# Autodesk Inventor assembly: Mark2
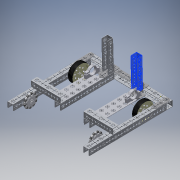
[picture p0: Inventor's stored thumbnail of the model, 180x180]
Saved by Autodesk Inventor 2017 (Build 210142000, 142)
## iProperties
Created: 2016-09-25
Part Number: Mark2
Document SubType Name: Assembly
Designer: Spartacles
Author: Spartacles
## Documents named in this file (14)
- C:\Users\Spartacles\Desktop\2016-Robot\2016launcher\Mark2.iam
- C:\Users\Spartacles\Desktop\2016-Robot\2016launcher\UTubes\Star3Tube.ipt
- C:\Users\Spartacles\Desktop\2016-Robot\2016launcher\UTubes\Star5Tube.ipt
- C:\Users\Spartacles\Desktop\2016-Robot\2016launcher\UTubes\Star7Tube.ipt
- C:\Users\Spartacles\Desktop\2016-Robot\Axle Hub\Axle hub thin.ipt
- C:\Users\Spartacles\Desktop\2016-Robot\Axel\Axel.ipt
- C:\Users\Spartacles\Desktop\2016-Robot\BlackWheels\4 Inch Wheel.ipt
- C:\Users\Spartacles\Desktop\2016-Robot\omni\3inch OmniWheel.iam
- C:\Users\Spartacles\Documents\Pitsco Education-739273\Pitsco Education-739273.ipt
- C:\Users\Spartacles\Documents\Pitsco Education-739272 (1)\Pitsco Education-739272.ipt
- C:\Users\Spartacles\Documents\Pitsco Education-739073\Pitsco Education-739073.ipt
- C:\Users\Spartacles\Desktop\2016-Robot\Angle brackets\User Library-739281 TETRIX Inside Corner Bracket.ipt
- C:\Users\Spartacles\Desktop\2016-Robot\Motor Mount\Tetrix Motor Mount.ipt
- C:\Users\Spartacles\Desktop\2016-Robot\Utubes\Utube_3.ipt
## Components (44 placed, 13 different names)
1. Star5Tube:1 — Mate:6, Flush:12, Flush:13, Mate:74, Mate:75, Mate:76, Mate:105, Mate:106, Mate:107, Mate:126, Mate:127, Mate:128
2. Star5Tube:2 — Flush:7, Flush:8, Mate:61, Mate:79, Mate:81, Mate:94, Mate:108, Mate:109, Mate:110, Mate:123, Mate:124, Mate:125
3. Star7Tube:1 — Mate:4, Flush:6, Flush:9, Mate:17, Mate:18, Mate:20, Mate:24, Mate:25, Mate:32, Mate:44, Flush:26, Mate:64, Mate:65, Mate:66
4. Star7Tube:2 — Flush:11, Flush:14, Mate:8, Mate:9, Mate:13, Mate:30, Mate:31, Mate:33, Mate:36, Mate:45, Mate:67, Mate:70, Mate:71
5. Star3Tube:1 — Mate:4, Flush:6, Flush:7, Flush:8, Flush:9, Mate:44, Flush:26, Mate:61
6. Star3Tube:2 — Mate:6, Flush:11, Flush:12, Flush:13, Flush:14, Mate:36, Mate:45
7. Axle hub thin:1 — Mate:19, Mate:20
8. Axle hub thin:2 — Mate:14, Mate:15, Mate:16, Mate:18
9. Axle hub thin:3 — Mate:12, Mate:13
10. Axle hub thin:4 — Mate:7, Mate:8, Mate:9, Mate:10, Mate:11
11. Axel:1 — Mate:16, Flush:16, Mate:17, Mate:19
12. Axel:2 — Mate:27, Flush:18, Mate:30, Mate:34, Mate:145, Mate:146
13. Axel:3 — Mate:23, Flush:17, Mate:26, Mate:141, Mate:142
14. Axel:4 — Mate:7, Flush:15, Mate:12
15. 4 Inch Wheel:1 — Mate:21, Mate:22, Flush:17
16. 4 Inch Wheel:2 — Mate:28, Mate:29, Flush:18
17. 3inch OmniWheel:1 [sub-assembly] — Mate:10, Mate:11, Flush:15
18. 3inch OmniWheel:2 [sub-assembly] — Mate:14, Mate:15, Flush:16
19. Axle hub thin:5 — Mate:21, Mate:22, Mate:23, Mate:24, Mate:32
20. Axle hub thin:6 — Mate:25, Mate:26
21. Axle hub thin:7 — Mate:27, Mate:28, Mate:29, Mate:31
22. Axle hub thin:8 — Mate:33, Mate:34
23. Star3Tube:3 — Mate:98, Mate:99, Mate:100, Mate:101, Mate:102, Mate:103, Mate:113, Mate:114, Mate:116, Mate:118, Mate:119
24. Star5Tube:3 — Mate:95, Mate:96, Mate:97, Mate:104, Mate:111, Mate:115, Mate:121
25. Pitsco Education-739273:1 — Mate:67, Mate:70, Mate:71, Mate:95, Mate:96
26. Pitsco Education-739273:2 — Mate:79, Mate:81, Mate:94, Mate:98, Mate:100, Mate:112
27. Pitsco Education-739273:3 — Mate:74, Mate:75, Mate:76, Mate:97, Mate:120, Mate:122
28. Pitsco Education-739273:4 — Mate:64, Mate:65, Mate:66, Mate:99
29. Pitsco Education-739272:1 — Mate:111, Mate:112, Mate:113, Mate:114, Mate:115, Mate:116, Mate:117
30. Pitsco Education-739272:2 — Mate:101, Mate:102, Mate:103, Mate:104
31. Pitsco Education-739073:1 — Mate:108, Mate:109, Mate:110, Mate:134
32. Pitsco Education-739073:3 — Mate:105, Mate:106, Mate:107, Mate:131
33. User Library-739281 TETRIX Inside Corner Bracket:1 — Mate:120, Mate:121, Mate:122, Mate:135, Mate:136, Mate:137
34. User Library-739281 TETRIX Inside Corner Bracket:2 — Mate:117, Mate:118, Mate:119, Mate:138, Mate:139, Mate:140
35. User Library-739281 TETRIX Inside Corner Bracket:3 — Mate:126, Mate:127, Mate:128, Mate:129, Mate:130
36. User Library-739281 TETRIX Inside Corner Bracket:4 — Mate:123, Mate:124, Mate:125, Mate:132, Mate:133
37. Tetrix Motor Mount:1 — Mate:129, Mate:130, Mate:131
38. Tetrix Motor Mount:2 — Mate:132, Mate:133, Mate:134
39. Utube_3:1 — Mate:138, Mate:139, Mate:140
40. Utube_3:2 — Mate:135, Mate:136, Mate:137
41. Axel:5 — Mate:141, Mate:142, Mate:143, Mate:144
42. Axel:6 — Mate:143, Mate:144
43. Axel:7 — Mate:145, Mate:146, Mate:147, Mate:148
44. Axel:8 — Mate:147, Mate:148
## Relationships (114: Mate 101, Flush 13)
- Mate:4: Star7Tube:1 ↔ Star3Tube:1
- Flush:6: Star7Tube:1 ↔ Star3Tube:1
- Flush:7: Star5Tube:2 ↔ Star3Tube:1
- Flush:8: Star5Tube:2 ↔ Star3Tube:1
- Flush:9: Star7Tube:1 ↔ Star3Tube:1
- Mate:6: Star5Tube:1 ↔ Star3Tube:2
- Flush:11: Star7Tube:2 ↔ Star3Tube:2
- Flush:12: Star5Tube:1 ↔ Star3Tube:2
- Flush:13: Star5Tube:1 ↔ Star3Tube:2
- Flush:14: Star7Tube:2 ↔ Star3Tube:2
- Mate:7: Axle hub thin:4 ↔ Axel:4
- Mate:8: Star7Tube:2 ↔ Axle hub thin:4
- Mate:9: Star7Tube:2 ↔ Axle hub thin:4
- Mate:10: Axle hub thin:4 ↔ 3inch OmniWheel:1
- Mate:11: Axle hub thin:4 ↔ 3inch OmniWheel:1
- Flush:15: Axel:4 ↔ 3inch OmniWheel:1
- Mate:12: Axle hub thin:3 ↔ Axel:4
- Mate:13: Star7Tube:2 ↔ Axle hub thin:3
- Mate:14: Axle hub thin:2 ↔ 3inch OmniWheel:2
- Mate:15: Axle hub thin:2 ↔ 3inch OmniWheel:2
- Mate:16: Axle hub thin:2 ↔ Axel:1
- Flush:16: Axel:1 ↔ 3inch OmniWheel:2
- Mate:17: Star7Tube:1 ↔ Axel:1
- Mate:18: Star7Tube:1 ↔ Axle hub thin:2
- Mate:19: Axle hub thin:1 ↔ Axel:1
- Mate:20: Star7Tube:1 ↔ Axle hub thin:1
- Mate:21: 4 Inch Wheel:1 ↔ Axle hub thin:5
- Mate:22: 4 Inch Wheel:1 ↔ Axle hub thin:5
- Mate:23: Axel:3 ↔ Axle hub thin:5
- Flush:17: Axel:3 ↔ 4 Inch Wheel:1
- Mate:24: Star7Tube:1 ↔ Axle hub thin:5
- Mate:25: Star7Tube:1 ↔ Axle hub thin:6
- Mate:26: Axel:3 ↔ Axle hub thin:6
- Mate:27: Axel:2 ↔ Axle hub thin:7
- Mate:28: 4 Inch Wheel:2 ↔ Axle hub thin:7
- Mate:29: 4 Inch Wheel:2 ↔ Axle hub thin:7
- Flush:18: Axel:2 ↔ 4 Inch Wheel:2
- Mate:30: Star7Tube:2 ↔ Axel:2
- Mate:31 (6.35 mm): Star7Tube:2 ↔ Axle hub thin:7
- Mate:32 (6.35 mm): Star7Tube:1 ↔ Axle hub thin:5
- Mate:33: Star7Tube:2 ↔ Axle hub thin:8
- Mate:34: Axel:2 ↔ Axle hub thin:8
- Mate:36: Star7Tube:2 ↔ Star3Tube:2
- Mate:44: Star7Tube:1 ↔ Star3Tube:1
- Flush:26: Star7Tube:1 ↔ Star3Tube:1
- Mate:45: Star7Tube:2 ↔ Star3Tube:2
- Mate:52 (0.2794 mm)
- Mate:61: Star5Tube:2 ↔ Star3Tube:1
- Mate:64: Star7Tube:1 ↔ Pitsco Education-739273:4
- Mate:65: Star7Tube:1 ↔ Pitsco Education-739273:4
- Mate:66: Star7Tube:1 ↔ Pitsco Education-739273:4
- Mate:67: Star7Tube:2 ↔ Pitsco Education-739273:1
- Mate:70: Star7Tube:2 ↔ Pitsco Education-739273:1
- Mate:71: Star7Tube:2 ↔ Pitsco Education-739273:1
- Mate:74: Star5Tube:1 ↔ Pitsco Education-739273:3
- Mate:75: Star5Tube:1 ↔ Pitsco Education-739273:3
- Mate:76: Star5Tube:1 ↔ Pitsco Education-739273:3
- Mate:79: Star5Tube:2 ↔ Pitsco Education-739273:2
- Mate:81: Star5Tube:2 ↔ Pitsco Education-739273:2
- Mate:94: Star5Tube:2 ↔ Pitsco Education-739273:2
- Mate:95: Star5Tube:3 ↔ Pitsco Education-739273:1
- Mate:96: Star5Tube:3 ↔ Pitsco Education-739273:1
- Mate:97: Star5Tube:3 ↔ Pitsco Education-739273:3
- Mate:98: Star3Tube:3 ↔ Pitsco Education-739273:2
- Mate:99: Star3Tube:3 ↔ Pitsco Education-739273:4
- Mate:100: Star3Tube:3 ↔ Pitsco Education-739273:2
- Mate:101: Star3Tube:3 ↔ Pitsco Education-739272:2
- Mate:102: Star3Tube:3 ↔ Pitsco Education-739272:2
- Mate:103: Star3Tube:3 ↔ Pitsco Education-739272:2
- Mate:104: Star5Tube:3 ↔ Pitsco Education-739272:2
- Mate:105: Star5Tube:1 ↔ Pitsco Education-739073:3
- Mate:106: Star5Tube:1 ↔ Pitsco Education-739073:3
- Mate:107: Star5Tube:1 ↔ Pitsco Education-739073:3
- Mate:108: Star5Tube:2 ↔ Pitsco Education-739073:1
- Mate:109: Star5Tube:2 ↔ Pitsco Education-739073:1
- Mate:110: Star5Tube:2 ↔ Pitsco Education-739073:1
- Mate:111: Star5Tube:3 ↔ Pitsco Education-739272:1
- Mate:112: Pitsco Education-739273:2 ↔ Pitsco Education-739272:1
- Mate:113: Star3Tube:3 ↔ Pitsco Education-739272:1
- Mate:114: Star3Tube:3 ↔ Pitsco Education-739272:1
- Mate:115: Star5Tube:3 ↔ Pitsco Education-739272:1
- Mate:116: Star3Tube:3 ↔ Pitsco Education-739272:1
- Mate:117 (2.0066 mm): Pitsco Education-739272:1 ↔ User Library-739281 TETRIX Inside Corner Bracket:2
- Mate:118: Star3Tube:3 ↔ User Library-739281 TETRIX Inside Corner Bracket:2
- Mate:119: Star3Tube:3 ↔ User Library-739281 TETRIX Inside Corner Bracket:2
- Mate:120: Pitsco Education-739273:3 ↔ User Library-739281 TETRIX Inside Corner Bracket:1
- Mate:121: Star5Tube:3 ↔ User Library-739281 TETRIX Inside Corner Bracket:1
- Mate:122: Pitsco Education-739273:3 ↔ User Library-739281 TETRIX Inside Corner Bracket:1
- Mate:123: Star5Tube:2 ↔ User Library-739281 TETRIX Inside Corner Bracket:4
- Mate:124: Star5Tube:2 ↔ User Library-739281 TETRIX Inside Corner Bracket:4
- Mate:125: Star5Tube:2 ↔ User Library-739281 TETRIX Inside Corner Bracket:4
- Mate:126: Star5Tube:1 ↔ User Library-739281 TETRIX Inside Corner Bracket:3
- Mate:127: Star5Tube:1 ↔ User Library-739281 TETRIX Inside Corner Bracket:3
- Mate:128: Star5Tube:1 ↔ User Library-739281 TETRIX Inside Corner Bracket:3
- Mate:129: User Library-739281 TETRIX Inside Corner Bracket:3 ↔ Tetrix Motor Mount:1
- Mate:130: User Library-739281 TETRIX Inside Corner Bracket:3 ↔ Tetrix Motor Mount:1
- Mate:131: Pitsco Education-739073:3 ↔ Tetrix Motor Mount:1
- Mate:132: User Library-739281 TETRIX Inside Corner Bracket:4 ↔ Tetrix Motor Mount:2
- Mate:133: User Library-739281 TETRIX Inside Corner Bracket:4 ↔ Tetrix Motor Mount:2
- Mate:134: Pitsco Education-739073:1 ↔ Tetrix Motor Mount:2
- Mate:135: User Library-739281 TETRIX Inside Corner Bracket:1 ↔ Utube_3:2
- Mate:136: User Library-739281 TETRIX Inside Corner Bracket:1 ↔ Utube_3:2
- Mate:137: User Library-739281 TETRIX Inside Corner Bracket:1 ↔ Utube_3:2
- Mate:138: User Library-739281 TETRIX Inside Corner Bracket:2 ↔ Utube_3:1
- Mate:139: User Library-739281 TETRIX Inside Corner Bracket:2 ↔ Utube_3:1
- Mate:140: User Library-739281 TETRIX Inside Corner Bracket:2 ↔ Utube_3:1
- Mate:141: Axel:3 ↔ Axel:5
- Mate:142: Axel:3 ↔ Axel:5
- Mate:143: Axel:5 ↔ Axel:6
- Mate:144: Axel:5 ↔ Axel:6
- Mate:145: Axel:2 ↔ Axel:7
- Mate:146: Axel:2 ↔ Axel:7
- Mate:147: Axel:7 ↔ Axel:8
- Mate:148: Axel:7 ↔ Axel:8
